# Autodesk Inventor assembly: Servo Mechanism
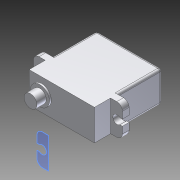
[picture p0: Inventor's stored thumbnail of the model, 180x180]
Saved by Autodesk Inventor 2014 SP1 (Build 180222100, 222)
## iProperties
Created: 2013-12-25
Part Number: Servo Mechanism
Document SubType Name: Assembly
Designer: tom
Author: tom
## Documents named in this file (3)
- C:\Users\tom\Documents\GitHub\Delta_Robots\Delatabot - Small Model\Inventor\Deltabot - Small Model\Servo Mechanism.iam
- C:\Users\tom\Documents\GitHub\Delta_Robots\Delatabot - Small Model\Inventor\Deltabot - Small Model\Component2.ipt
- C:\Users\tom\Documents\GitHub\Boat_Bot\Servo Bracket.ipt
## Components (2 placed, 2 different names)
1. Servo — Flush:1
2. Servo Bracket:1 — Flush:1
## Relationships (1: Flush 1)
- Flush:1: Servo ↔ Servo Bracket:1
